# Autodesk Inventor assembly: 2 Pin Male
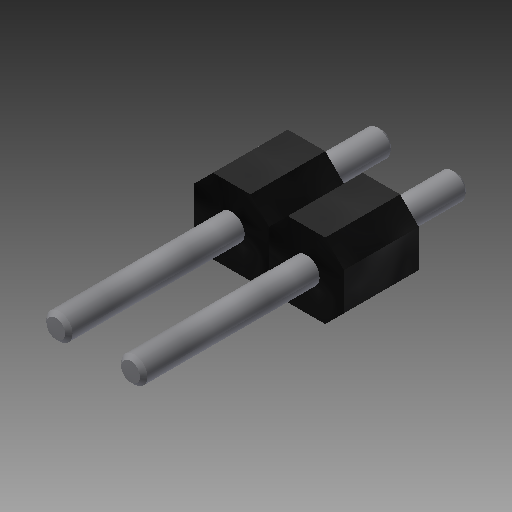
[picture p0: Inventor's stored thumbnail of the model, 512x512]
Saved by Autodesk Inventor 2017 (Build 210142000, 142)
## iProperties
Created: 2016-08-11
Part Number: 2 Pin Male
Document SubType Name: Assembly
Designer: ge937963
Author: ge937963
## Documents named in this file (2)
- Z:\allusers\Diagnostics\Inventor Files\3dPrintedPCR\2 Pin Male.iam
- Z:\allusers\Diagnostics\Inventor Files\3dPrintedPCR\Pin.ipt
## Components (2 placed, 1 different names)
1. Pin:1 — Flush:1, Flush:2, Mate:1
2. Pin:2 — Flush:1, Flush:2, Mate:1
## Relationships (3: Flush 2, Mate 1)
- Flush:1: Pin:1 ↔ Pin:2
- Flush:2: Pin:1 ↔ Pin:2
- Mate:1: Pin:1 ↔ Pin:2
